# Autodesk Inventor assembly: MONTAGEM INTAKE v2
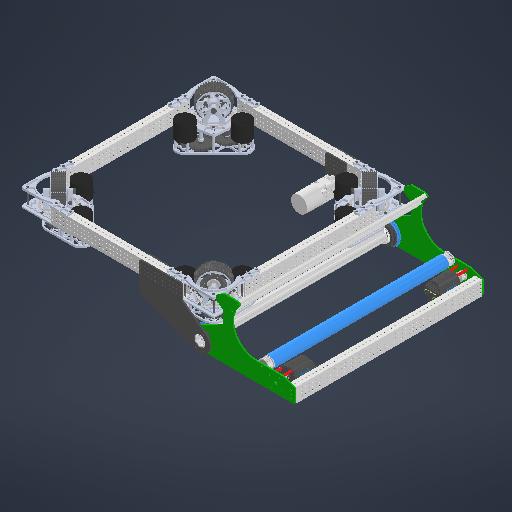
[picture p0: Inventor's stored thumbnail of the model, 512x512]
Saved by Autodesk Inventor 2026 (Build 300175000, 175)
## iProperties
Created: 2026-06-18
Part Number: MONTAGEM INTAKE v2
Document SubType Name: Assembly
Designer: DELL
Author: DELL
## Documents named in this file (24)
- C:\Users\DELL\OneDrive - SFIEMT\Área de Trabalho\PROJETO FRC\CAD\MONTAGEM INTAKE v2.iam
- C:\Users\DELL\OneDrive - SFIEMT\Área de Trabalho\PROJETO FRC\CAD\CHASSI.iam
- C:\Users\DELL\OneDrive - SFIEMT\Área de Trabalho\PROJETO FRC\CAD\INTAKE\TUBO MAXSPLINE.ipt
- C:\Users\DELL\OneDrive - SFIEMT\Área de Trabalho\PROJETO FRC\CAD\INTAKE\ROLAMENTO MAXSPLINE.iam
- C:\Users\DELL\OneDrive - SFIEMT\Área de Trabalho\PROJETO FRC\CAD\INTAKE\MOTOR NEO.iam
- C:\Users\DELL\OneDrive - SFIEMT\Área de Trabalho\PROJETO FRC\CAD\INTAKE\COROA 40T.ipt
- C:\Users\DELL\OneDrive - SFIEMT\Área de Trabalho\PROJETO FRC\CAD\INTAKE\COROA 14T.ipt
- C:\Users\DELL\OneDrive - SFIEMT\Área de Trabalho\PROJETO FRC\CAD\INTAKE\CHAPA FIXAÇÃO ESQUERDA 1 V2.ipt
- C:\Users\DELL\OneDrive - SFIEMT\Área de Trabalho\PROJETO FRC\CAD\INTAKE\CHAPA FIXAÇÃO ESQUERDA 2.ipt
- C:\Users\DELL\OneDrive - SFIEMT\Área de Trabalho\PROJETO FRC\CAD\INTAKE\EIXO SEXTAVADO MOTOR.ipt
- C:\Users\DELL\OneDrive - SFIEMT\Área de Trabalho\PROJETO FRC\CAD\INTAKE\ROLAMENTO SEXTAVADO.ipt
- C:\Users\DELL\OneDrive - SFIEMT\Área de Trabalho\PROJETO FRC\CAD\INTAKE\CHAPA FIXAÇÃO DIREITA 1 V2.ipt
- C:\Users\DELL\OneDrive - SFIEMT\Área de Trabalho\PROJETO FRC\CAD\INTAKE\CHAPA FIXAÇÃO DIREITA 2.ipt
- C:\Users\DELL\OneDrive - SFIEMT\Área de Trabalho\PROJETO FRC\CAD\INTAKE\CHAPA LATERAL INTAKE V2.ipt
- C:\Users\DELL\OneDrive - SFIEMT\Área de Trabalho\PROJETO FRC\CAD\INTAKE\KRAKEN X60.ipt
- C:\Users\DELL\OneDrive - SFIEMT\Área de Trabalho\PROJETO FRC\CAD\INTAKE\ADAPTADOR EIXO KRAKEN.ipt
- C:\Users\DELL\OneDrive - SFIEMT\Área de Trabalho\PROJETO FRC\CAD\INTAKE\POLIA 15D.ipt
- C:\Users\DELL\OneDrive - SFIEMT\Área de Trabalho\PROJETO FRC\CAD\INTAKE\PERFIL 50X25 STEMOS 661,4MM.ipt
- C:\Users\DELL\OneDrive - SFIEMT\Área de Trabalho\PROJETO FRC\CAD\INTAKE\Acoplador de tubo.ipt
- C:\Users\DELL\OneDrive - SFIEMT\Área de Trabalho\PROJETO FRC\CAD\INTAKE\EIXO SEXTAVADO 661,4MM.ipt
- C:\Users\DELL\OneDrive - SFIEMT\Área de Trabalho\PROJETO FRC\CAD\INTAKE\POLIA 23D ROLETE.ipt
- C:\Users\DELL\OneDrive - SFIEMT\Área de Trabalho\PROJETO FRC\CAD\INTAKE\TUBO.ipt
- C:\Users\DELL\OneDrive - SFIEMT\Área de Trabalho\PROJETO FRC\CAD\INTAKE\ESPAÇADOR.ipt
- C:\Users\DELL\OneDrive - SFIEMT\Área de Trabalho\PROJETO FRC\CAD\INTAKE\PRESILHA MAXSPLINE.iam
## Components (45 placed, 23 different names)
1. CHASSI:1 [sub-assembly] — Coincidente:4, Coincidente:5, Coincidente:6, Alinhado:1, Alinhado:2, Alinhado:3, Alinhado:4, Alinhado:5, Coincidente:10, Coincidente:11, Coincidente:22, Coincidente:23, Coincidente:24, Coincidente:25, Coincidente:26, Coincidente:27
2. TUBO MAXSPLINE:1 — Coincidente:12, Coincidente:13, Coincidente:14, Coincidente:34, Coincidente:37, Coincidente:44, Coincidente:102, Coincidente:103, Coincidente:105, Coincidente:108
3. ROLAMENTO MAXSPLINE:1 [sub-assembly] — Alinhado:3, Alinhado:4, Alinhado:5, Coincidente:9, Alinhado:6, Coincidente:12
4. ROLAMENTO MAXSPLINE:2 [sub-assembly] — Coincidente:8, Coincidente:9, Alinhado:6, Coincidente:106
5. ROLAMENTO MAXSPLINE:3 [sub-assembly] — Coincidente:31, Coincidente:32, Coincidente:33, Coincidente:104
6. ROLAMENTO MAXSPLINE:4 [sub-assembly] — Coincidente:28, Coincidente:29, Coincidente:30
7. MOTOR NEO:1 [sub-assembly] — Coincidente:7, Alinhado:1, Alinhado:2
8. COROA 40T:1 — Coincidente:34, Coincidente:36, Coincidente:43, Coincidente:45, Coincidente:46
9. COROA 40T:2 — Coincidente:13, Coincidente:14, Coincidente:15, Coincidente:38, Coincidente:39, Coincidente:43
10. COROA 14T:1 — Coincidente:17, Coincidente:18, Coincidente:19, Coincidente:109
11. CHAPA FIXAÇÃO ESQUERDA 2:1 — Coincidente:4, Coincidente:5, Coincidente:6, Coincidente:7, Coincidente:8, Coincidente:15, Coincidente:17, Coincidente:107
12. EIXO SEXTAVADO MOTOR:1 — Coincidente:18, Coincidente:19, Alinhado:11, Coincidente:112
13. ROLAMENTO SEXTAVADO:1 — Coincidente:110, Coincidente:111, Coincidente:112
14. CHAPA FIXAÇÃO DIREITA 1 V2:1 — Coincidente:25, Coincidente:26, Coincidente:27, Coincidente:28, Coincidente:29, Coincidente:30
15. CHAPA FIXAÇÃO DIREITA 2:1 — Coincidente:22, Coincidente:23, Coincidente:24, Coincidente:31, Coincidente:32, Coincidente:33, Coincidente:36
16. KRAKEN X60:1 — Coincidente:40, Coincidente:41, Coincidente:42, Coincidente:51, Coincidente:59, Coincidente:97, Coincidente:98, Coincidente:100, Coincidente:101
17. CHAPA LATERAL INTAKE V2:1 — Coincidente:37, Coincidente:38, Coincidente:39, Coincidente:40, Coincidente:41, Coincidente:42, Coincidente:55, Coincidente:58, Coincidente:66, Coincidente:67, Coincidente:68, Coincidente:69, Coincidente:70, Coincidente:71, Coincidente:72, Coincidente:73, Coincidente:74, Coincidente:80, Coincidente:81, Coincidente:93, Coincidente:94, Coincidente:95, Coincidente:96
18. CHAPA LATERAL INTAKE V2:2 — Coincidente:44, Coincidente:45, Coincidente:46, Coincidente:47, Coincidente:48, Coincidente:49, Coincidente:56, Coincidente:82, Coincidente:85, Coincidente:87, Coincidente:89, Coincidente:91
19. KRAKEN X60:2 — Coincidente:47, Coincidente:48, Coincidente:49, Coincidente:50, Coincidente:54, Coincidente:86, Coincidente:88, Coincidente:90, Coincidente:92
20. ADAPTADOR EIXO KRAKEN:1 — Coincidente:51, Coincidente:55
21. ADAPTADOR EIXO KRAKEN:2 — Coincidente:50, Alinhado:9
22. POLIA 15D:1 — Coincidente:54, Alinhado:9, Coincidente:56
23. POLIA 15D:2 — Coincidente:58, Coincidente:59
24. PERFIL 50X25 STEMOS 661,4MM:1 — Coincidente:60, Coincidente:61, Coincidente:62, Coincidente:63, Coincidente:64, Coincidente:65, Coincidente:68
25. Acoplador de tubo:1 — Coincidente:60, Coincidente:61, Coincidente:62, Coincidente:66, Coincidente:67
26. Acoplador de tubo:2 — Coincidente:63, Coincidente:64, Coincidente:65
27. EIXO SEXTAVADO 661,4MM:1 — Coincidente:69, Coincidente:70
28. EIXO SEXTAVADO 661,4MM:2 — Coincidente:71, Coincidente:72
29. EIXO SEXTAVADO 661,4MM:3 — Coincidente:73, Coincidente:74
30. POLIA 23D ROLETE:1 — Coincidente:77, Coincidente:78, Coincidente:79, Coincidente:82, Coincidente:83, Coincidente:84
31. POLIA 23D ROLETE:2 — Coincidente:75, Coincidente:76, Coincidente:79, Coincidente:80, Coincidente:81
32. ROLAMENTO SEXTAVADO:2 — Coincidente:77, Coincidente:78
33. ROLAMENTO SEXTAVADO:3 — Coincidente:75, Coincidente:76
34. TUBO:1 — Coincidente:83, Coincidente:84
35. ESPAÇADOR:1 — Coincidente:85, Coincidente:86
36. ESPAÇADOR:2 — Coincidente:91, Coincidente:92
37. ESPAÇADOR:5 — Coincidente:93, Coincidente:100
38. ESPAÇADOR:6 — Coincidente:87, Coincidente:88
39. ESPAÇADOR:7 — Coincidente:89, Coincidente:90
40. ESPAÇADOR:8 — Coincidente:94, Coincidente:101
41. ESPAÇADOR:10 — Coincidente:95, Coincidente:98
42. ESPAÇADOR:11 — Coincidente:96, Coincidente:97
43. PRESILHA MAXSPLINE:1 [sub-assembly] — Coincidente:105, Alinhado:10, Coincidente:106
44. PRESILHA MAXSPLINE:2 [sub-assembly] — Coincidente:102, Coincidente:103, Coincidente:104, Alinhado:10
45. CHAPA FIXAÇÃO ESQUERDA 1 V2:1 — Coincidente:107, Coincidente:108, Coincidente:109, Coincidente:110, Coincidente:111, Alinhado:11
## Relationships (110: Mate 101, Flush 9)
- Coincidente:4 [Mate]: CHASSI:1 ↔ CHAPA FIXAÇÃO ESQUERDA 2:1
- Coincidente:5 [Mate]: CHASSI:1 ↔ CHAPA FIXAÇÃO ESQUERDA 2:1
- Coincidente:6 [Mate]: CHASSI:1 ↔ CHAPA FIXAÇÃO ESQUERDA 2:1
- Coincidente:7 [Mate]: MOTOR NEO:1 ↔ CHAPA FIXAÇÃO ESQUERDA 2:1
- Alinhado:1 [Flush] (205 mm): CHASSI:1 ↔ MOTOR NEO:1
- Alinhado:2 [Flush] (55 mm): CHASSI:1 ↔ MOTOR NEO:1
- Alinhado:3 [Flush]: CHASSI:1 ↔ ROLAMENTO MAXSPLINE:1
- Alinhado:4 [Flush] (17 mm): CHASSI:1 ↔ ROLAMENTO MAXSPLINE:1
- Alinhado:5 [Flush] (113 mm): CHASSI:1 ↔ ROLAMENTO MAXSPLINE:1
- Coincidente:8 [Mate]: ROLAMENTO MAXSPLINE:2 ↔ CHAPA FIXAÇÃO ESQUERDA 2:1
- Coincidente:9 [Mate]: ROLAMENTO MAXSPLINE:1 ↔ ROLAMENTO MAXSPLINE:2
- Alinhado:6 [Flush]: ROLAMENTO MAXSPLINE:1 ↔ ROLAMENTO MAXSPLINE:2
- Coincidente:10 [Mate]: CHASSI:1
- Coincidente:11 [Mate]: CHASSI:1
- Coincidente:12 [Mate]: TUBO MAXSPLINE:1 ↔ ROLAMENTO MAXSPLINE:1
- Coincidente:13 [Mate]: TUBO MAXSPLINE:1 ↔ COROA 40T:2
- Coincidente:14 [Mate]: TUBO MAXSPLINE:1 ↔ COROA 40T:2
- Coincidente:15 [Mate] (0.5 mm): COROA 40T:2 ↔ CHAPA FIXAÇÃO ESQUERDA 2:1
- Coincidente:17 [Mate] (0.5 mm): COROA 14T:1 ↔ CHAPA FIXAÇÃO ESQUERDA 2:1
- Coincidente:18 [Mate]: COROA 14T:1 ↔ EIXO SEXTAVADO MOTOR:1
- Coincidente:19 [Mate]: COROA 14T:1 ↔ EIXO SEXTAVADO MOTOR:1
- Coincidente:22 [Mate]: CHASSI:1 ↔ CHAPA FIXAÇÃO DIREITA 2:1
- Coincidente:23 [Mate]: CHASSI:1 ↔ CHAPA FIXAÇÃO DIREITA 2:1
- Coincidente:24 [Mate]: CHASSI:1 ↔ CHAPA FIXAÇÃO DIREITA 2:1
- Coincidente:25 [Mate]: CHASSI:1 ↔ CHAPA FIXAÇÃO DIREITA 1 V2:1
- Coincidente:26 [Mate]: CHASSI:1 ↔ CHAPA FIXAÇÃO DIREITA 1 V2:1
- Coincidente:27 [Mate]: CHASSI:1 ↔ CHAPA FIXAÇÃO DIREITA 1 V2:1
- Coincidente:28 [Mate]: ROLAMENTO MAXSPLINE:4 ↔ CHAPA FIXAÇÃO DIREITA 1 V2:1
- Coincidente:29 [Mate]: ROLAMENTO MAXSPLINE:4 ↔ CHAPA FIXAÇÃO DIREITA 1 V2:1
- Coincidente:30 [Mate]: ROLAMENTO MAXSPLINE:4 ↔ CHAPA FIXAÇÃO DIREITA 1 V2:1
- Coincidente:31 [Mate]: ROLAMENTO MAXSPLINE:3 ↔ CHAPA FIXAÇÃO DIREITA 2:1
- Coincidente:32 [Mate]: ROLAMENTO MAXSPLINE:3 ↔ CHAPA FIXAÇÃO DIREITA 2:1
- Coincidente:33 [Mate]: ROLAMENTO MAXSPLINE:3 ↔ CHAPA FIXAÇÃO DIREITA 2:1
- Coincidente:34 [Mate]: TUBO MAXSPLINE:1 ↔ COROA 40T:1
- Coincidente:36 [Mate] (0.5 mm): COROA 40T:1 ↔ CHAPA FIXAÇÃO DIREITA 2:1
- Coincidente:37 [Mate]: TUBO MAXSPLINE:1 ↔ CHAPA LATERAL INTAKE V2:1
- Coincidente:38 [Mate]: COROA 40T:2 ↔ CHAPA LATERAL INTAKE V2:1
- Coincidente:39 [Mate]: COROA 40T:2 ↔ CHAPA LATERAL INTAKE V2:1
- Coincidente:40 [Mate]: KRAKEN X60:1 ↔ CHAPA LATERAL INTAKE V2:1
- Coincidente:41 [Mate]: KRAKEN X60:1 ↔ CHAPA LATERAL INTAKE V2:1
- Coincidente:42 [Mate]: KRAKEN X60:1 ↔ CHAPA LATERAL INTAKE V2:1
- Coincidente:43 [Mate]: COROA 40T:1 ↔ COROA 40T:2
- Coincidente:44 [Mate]: TUBO MAXSPLINE:1 ↔ CHAPA LATERAL INTAKE V2:2
- Coincidente:45 [Mate]: COROA 40T:1 ↔ CHAPA LATERAL INTAKE V2:2
- Coincidente:46 [Mate]: COROA 40T:1 ↔ CHAPA LATERAL INTAKE V2:2
- Coincidente:47 [Mate]: CHAPA LATERAL INTAKE V2:2 ↔ KRAKEN X60:2
- Coincidente:48 [Mate]: CHAPA LATERAL INTAKE V2:2 ↔ KRAKEN X60:2
- Coincidente:49 [Mate]: CHAPA LATERAL INTAKE V2:2 ↔ KRAKEN X60:2
- Coincidente:50 [Mate]: KRAKEN X60:2 ↔ ADAPTADOR EIXO KRAKEN:2
- Coincidente:51 [Mate]: KRAKEN X60:1 ↔ ADAPTADOR EIXO KRAKEN:1
- Coincidente:54 [Mate]: KRAKEN X60:2 ↔ POLIA 15D:1
- Alinhado:9 [Flush]: ADAPTADOR EIXO KRAKEN:2 ↔ POLIA 15D:1
- Coincidente:55 [Mate] (1 mm): CHAPA LATERAL INTAKE V2:1 ↔ ADAPTADOR EIXO KRAKEN:1
- Coincidente:56 [Mate] (1 mm): CHAPA LATERAL INTAKE V2:2 ↔ POLIA 15D:1
- Coincidente:58 [Mate] (1 mm): CHAPA LATERAL INTAKE V2:1 ↔ POLIA 15D:2
- Coincidente:59 [Mate]: KRAKEN X60:1 ↔ POLIA 15D:2
- Coincidente:60 [Mate] (1.3 mm): PERFIL 50X25 STEMOS 661,4MM:1 ↔ Acoplador de tubo:1
- Coincidente:61 [Mate] (1.3 mm): PERFIL 50X25 STEMOS 661,4MM:1 ↔ Acoplador de tubo:1
- Coincidente:62 [Mate]: PERFIL 50X25 STEMOS 661,4MM:1 ↔ Acoplador de tubo:1
- Coincidente:63 [Mate] (1.3 mm): PERFIL 50X25 STEMOS 661,4MM:1 ↔ Acoplador de tubo:2
- Coincidente:64 [Mate] (1.3 mm): PERFIL 50X25 STEMOS 661,4MM:1 ↔ Acoplador de tubo:2
- Coincidente:65 [Mate]: PERFIL 50X25 STEMOS 661,4MM:1 ↔ Acoplador de tubo:2
- Coincidente:66 [Mate]: CHAPA LATERAL INTAKE V2:1 ↔ Acoplador de tubo:1
- Coincidente:67 [Mate]: CHAPA LATERAL INTAKE V2:1 ↔ Acoplador de tubo:1
- Coincidente:68 [Mate]: CHAPA LATERAL INTAKE V2:1 ↔ PERFIL 50X25 STEMOS 661,4MM:1
- Coincidente:69 [Mate]: CHAPA LATERAL INTAKE V2:1 ↔ EIXO SEXTAVADO 661,4MM:1
- Coincidente:70 [Mate]: CHAPA LATERAL INTAKE V2:1 ↔ EIXO SEXTAVADO 661,4MM:1
- Coincidente:71 [Mate]: CHAPA LATERAL INTAKE V2:1 ↔ EIXO SEXTAVADO 661,4MM:2
- Coincidente:72 [Mate]: CHAPA LATERAL INTAKE V2:1 ↔ EIXO SEXTAVADO 661,4MM:2
- Coincidente:73 [Mate]: CHAPA LATERAL INTAKE V2:1 ↔ EIXO SEXTAVADO 661,4MM:3
- Coincidente:74 [Mate]: CHAPA LATERAL INTAKE V2:1 ↔ EIXO SEXTAVADO 661,4MM:3
- Coincidente:75 [Mate]: POLIA 23D ROLETE:2 ↔ ROLAMENTO SEXTAVADO:3
- Coincidente:76 [Mate]: POLIA 23D ROLETE:2 ↔ ROLAMENTO SEXTAVADO:3
- Coincidente:77 [Mate]: POLIA 23D ROLETE:1 ↔ ROLAMENTO SEXTAVADO:2
- Coincidente:78 [Mate]: POLIA 23D ROLETE:1 ↔ ROLAMENTO SEXTAVADO:2
- Coincidente:79 [Mate]: POLIA 23D ROLETE:1 ↔ POLIA 23D ROLETE:2
- Coincidente:80 [Mate]: CHAPA LATERAL INTAKE V2:1 ↔ POLIA 23D ROLETE:2
- Coincidente:81 [Mate] (1 mm): CHAPA LATERAL INTAKE V2:1 ↔ POLIA 23D ROLETE:2
- Coincidente:82 [Mate]: CHAPA LATERAL INTAKE V2:2 ↔ POLIA 23D ROLETE:1
- Coincidente:83 [Mate]: POLIA 23D ROLETE:1 ↔ TUBO:1
- Coincidente:84 [Mate]: POLIA 23D ROLETE:1 ↔ TUBO:1
- Coincidente:85 [Mate]: CHAPA LATERAL INTAKE V2:2 ↔ ESPAÇADOR:1
- Coincidente:86 [Mate]: KRAKEN X60:2 ↔ ESPAÇADOR:1
- Coincidente:87 [Mate]: CHAPA LATERAL INTAKE V2:2 ↔ ESPAÇADOR:6
- Coincidente:88 [Mate]: KRAKEN X60:2 ↔ ESPAÇADOR:6
- Coincidente:89 [Mate]: CHAPA LATERAL INTAKE V2:2 ↔ ESPAÇADOR:7
- Coincidente:90 [Mate]: KRAKEN X60:2 ↔ ESPAÇADOR:7
- Coincidente:91 [Mate]: CHAPA LATERAL INTAKE V2:2 ↔ ESPAÇADOR:2
- Coincidente:92 [Mate]: KRAKEN X60:2 ↔ ESPAÇADOR:2
- Coincidente:93 [Mate]: CHAPA LATERAL INTAKE V2:1 ↔ ESPAÇADOR:5
- Coincidente:94 [Mate]: CHAPA LATERAL INTAKE V2:1 ↔ ESPAÇADOR:8
- Coincidente:95 [Mate]: CHAPA LATERAL INTAKE V2:1 ↔ ESPAÇADOR:10
- Coincidente:96 [Mate]: CHAPA LATERAL INTAKE V2:1 ↔ ESPAÇADOR:11
- Coincidente:97 [Mate]: KRAKEN X60:1 ↔ ESPAÇADOR:11
- Coincidente:98 [Mate]: KRAKEN X60:1 ↔ ESPAÇADOR:10
- Coincidente:100 [Mate]: KRAKEN X60:1 ↔ ESPAÇADOR:5
- Coincidente:101 [Mate]: KRAKEN X60:1 ↔ ESPAÇADOR:8
- Coincidente:102 [Mate]: TUBO MAXSPLINE:1 ↔ PRESILHA MAXSPLINE:2
- Coincidente:103 [Mate] (0.1 mm): TUBO MAXSPLINE:1 ↔ PRESILHA MAXSPLINE:2
- Coincidente:104 [Mate]: ROLAMENTO MAXSPLINE:3 ↔ PRESILHA MAXSPLINE:2
- Coincidente:105 [Mate]: TUBO MAXSPLINE:1 ↔ PRESILHA MAXSPLINE:1
- Alinhado:10 [Flush]: PRESILHA MAXSPLINE:1 ↔ PRESILHA MAXSPLINE:2
- Coincidente:106 [Mate]: ROLAMENTO MAXSPLINE:2 ↔ PRESILHA MAXSPLINE:1
- Coincidente:107 [Mate]: CHAPA FIXAÇÃO ESQUERDA 2:1 ↔ CHAPA FIXAÇÃO ESQUERDA 1 V2:1
- Coincidente:108 [Mate]: TUBO MAXSPLINE:1 ↔ CHAPA FIXAÇÃO ESQUERDA 1 V2:1
- Coincidente:109 [Mate]: COROA 14T:1 ↔ CHAPA FIXAÇÃO ESQUERDA 1 V2:1
- Coincidente:110 [Mate]: ROLAMENTO SEXTAVADO:1 ↔ CHAPA FIXAÇÃO ESQUERDA 1 V2:1
- Coincidente:111 [Mate]: ROLAMENTO SEXTAVADO:1 ↔ CHAPA FIXAÇÃO ESQUERDA 1 V2:1
- Alinhado:11 [Flush]: EIXO SEXTAVADO MOTOR:1 ↔ CHAPA FIXAÇÃO ESQUERDA 1 V2:1
- Coincidente:112 [Mate]: EIXO SEXTAVADO MOTOR:1 ↔ ROLAMENTO SEXTAVADO:1
